# Autodesk Inventor assembly: Zespół1
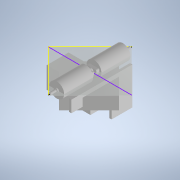
[picture p0: Inventor's stored thumbnail of the model, 180x180]
Saved by Autodesk Inventor 2020 (Build 240168000, 168)
## iProperties
Created: 2019-06-28
Part Number: Zespół1
Document SubType Name: Assembly
Designer: atmat
Author: atmat
## Documents named in this file (6)
- C:\Users\atmat\Documents\1.Projects\1.Roboty\1.Rainbow\1.Reincarnation\Czesci\Ver 2\Zespół1.iam
- C:\Users\atmat\Documents\1.Projects\1.Roboty\1.Rainbow\1.Reincarnation\Czesci\Ver 2\Silnik_SKUA.ipt
- C:\Users\atmat\Documents\1.Projects\1.Roboty\1.Rainbow\1.Reincarnation\Czesci\Ver 2\Platworma_10x10.ipt
- C:\Users\atmat\Documents\1.Projects\1.Roboty\1.Rainbow\1.Reincarnation\Czesci\Ver 2\Bateria_22V2.ipt
- C:\Users\atmat\Documents\1.Projects\1.Roboty\1.Rainbow\1.Reincarnation\Czesci\Ver 2\Bateria_22V2_Rozlozona.ipt
- C:\Users\atmat\Documents\1.Projects\1.Roboty\1.Rainbow\1.Reincarnation\Czesci\S5_Mainboard.ipt
## Components (6 placed, 5 different names)
1. Silnik_SKUA:1 — Zestawiające:1, Równoległe:1, Równoległe:2, Zestawiające:3, Zestawiające:4
2. Silnik_SKUA:2 — Zestawiające:1, Równoległe:1, Równoległe:2, Styczny:1
3. Platworma_10x10:1 — Zestawiające:3, Zestawiające:4, Zestawiające:6, Kątowe:1
4. Bateria_22V2:1 — Styczny:1, Kątowe:1, Równoległe:3, Zestawiające:7
5. Bateria_22V2_Rozlozona:1 — Równoległe:3
6. S5_Mainboard:1 — Zestawiające:7
## Relationships (10: Mate 5, Flush 3, Tangent 1, Angle 1)
- Zestawiające:1 [Mate]: Silnik_SKUA:1 ↔ Silnik_SKUA:2
- Równoległe:1 [Flush]: Silnik_SKUA:1 ↔ Silnik_SKUA:2
- Równoległe:2 [Flush]: Silnik_SKUA:1 ↔ Silnik_SKUA:2
- Zestawiające:3 [Mate]: Silnik_SKUA:1 ↔ Platworma_10x10:1
- Zestawiające:4 [Mate]: Silnik_SKUA:1 ↔ Platworma_10x10:1
- Zestawiające:6 [Mate]: Platworma_10x10:1
- Styczny:1 [Tangent]: Silnik_SKUA:2 ↔ Bateria_22V2:1
- Kątowe:1 [Angle] (0 deg): Platworma_10x10:1 ↔ Bateria_22V2:1
- Równoległe:3 [Flush]: Bateria_22V2:1 ↔ Bateria_22V2_Rozlozona:1
- Zestawiające:7 [Mate]: Bateria_22V2:1 ↔ S5_Mainboard:1
